# Autodesk Inventor assembly: TT_Tray
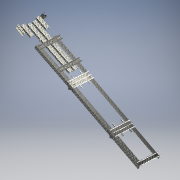
[picture p0: Inventor's stored thumbnail of the model, 180x180]
Saved by Autodesk Inventor 2019 (Build 230136000, 136)
## iProperties
Created: 2020-02-09
Part Number: TT_Tray
Document SubType Name: Assembly
Designer: samue
Author: samue
## Documents named in this file (25)
- C:\Users\samue\OneDrive\Desktop\CAD\TT_Tray.iam
- C:\Users\samue\OneDrive\Desktop\SID Library-20181221T043518Z-001\2018 BNS-VRC-SID Library\Structure\C-Channels\C-Channel 1x2x1\Aluminum C-Channel 1x2x1x30.ipt
- C:\Users\samue\OneDrive\Desktop\SID Library-20181221T043518Z-001\2018 BNS-VRC-SID Library\Structure\Standoffs _ Couplers\Standoff 0.50_.ipt
- C:\Users\samue\OneDrive\Desktop\SID Library-20181221T043518Z-001\2018 BNS-VRC-SID Library\Structure\C-Channels\C-Channel 1x2x1\Aluminum C-Channel 1x2x1x7.ipt
- C:\Users\samue\OneDrive\Desktop\SID Library-20181221T043518Z-001\2018 BNS-VRC-SID Library\Structure\C-Channels\C-Channel 1x2x1\Aluminum C-Channel 1x2x1x12.ipt
- C:\Users\samue\OneDrive\Desktop\SID Library-20181221T043518Z-001\2018 BNS-VRC-SID Library\Motion\Bearing Flat.ipt
- C:\Users\samue\OneDrive\Desktop\SID Library-20181221T043518Z-001\2018 BNS-VRC-SID Library\Structure\Screws _ Nuts\Screw 8-32 x 0.750_.ipt
- C:\Users\samue\OneDrive\Desktop\SID Library-20181221T043518Z-001\2018 BNS-VRC-SID Library\Structure\Screws _ Nuts\Screw 8-32 x 0.500_.ipt
- C:\Users\samue\OneDrive\Desktop\SID Library-20181221T043518Z-001\2018 BNS-VRC-SID Library\Structure\C-Channels\C-Channel 1x2x1\Aluminum C-Channel 1x2x1x5.ipt
- C:\Users\samue\OneDrive\Desktop\SID Library-20181221T043518Z-001\2018 BNS-VRC-SID Library\Structure\Screws _ Nuts\8-32 Nylon-Insert Thin Hex Locknut.iam
- C:\Users\samue\OneDrive\Desktop\SID Library-20181221T043518Z-001\2018 BNS-VRC-SID Library\Motion\Washers _ Spacers\Spacer (Nylon), 0.125_.ipt
- C:\Users\samue\OneDrive\Desktop\SID Library-20181221T043518Z-001\2018 BNS-VRC-SID Library\Motion\Washers _ Spacers\Washer, Steel, 0.032_.ipt
- C:\Users\samue\OneDrive\Desktop\SID Library-20181221T043518Z-001\2018 BNS-VRC-SID Library\Structure\Screws _ Nuts\Screw 8-32 x 1.250_.ipt
- C:\Users\samue\OneDrive\Desktop\SID Library-20181221T043518Z-001\2018 BNS-VRC-SID Library\Motion\Washers _ Spacers\Spacer (Nylon), 0.250_.ipt
- C:\Users\samue\OneDrive\Desktop\SID Library-20181221T043518Z-001\2018 BNS-VRC-SID Library\Structure\Screws _ Nuts\Screw 8-32 x 1.500_.ipt
- C:\Users\samue\OneDrive\Desktop\SID Library-20181221T043518Z-001\2018 BNS-VRC-SID Library\Structure\Screws _ Nuts\Nut 8-32 Keps.ipt
- C:\Users\samue\OneDrive\Desktop\SID Library-20181221T043518Z-001\2018 BNS-VRC-SID Library\Structure\Angles\Aluminum Angle\Aluminum Angle 2x2x25.ipt
- C:\Users\samue\OneDrive\Desktop\SID Library-20181221T043518Z-001\2018 BNS-VRC-SID Library\Motion\Washers _ Spacers\Spacer (Nylon), 0.500_.ipt
- C:\Users\samue\OneDrive\Desktop\SID Library-20181221T043518Z-001\2018 BNS-VRC-SID Library\Structure\Screws _ Nuts\8-32 Shoulder Screw.ipt
- C:\Users\samue\OneDrive\Desktop\SID Library-20181221T043518Z-001\2018 BNS-VRC-SID Library\Structure\Gussets\45 Degree Gusset.ipt
- C:\Users\samue\OneDrive\Desktop\SID Library-20181221T043518Z-001\2018 BNS-VRC-SID Library\Structure\Screws _ Nuts\Screw 8-32 x 0.375_.ipt
- C:\Users\samue\OneDrive\Desktop\SID Library-20181221T043518Z-001\2018 BNS-VRC-SID Library\Structure\C-Channels\C-Channel 1x2x1\Aluminum C-Channel 1x2x1x13.ipt
- C:\Users\samue\OneDrive\Desktop\SID Library-20181221T043518Z-001\2018 BNS-VRC-SID Library\Structure\Angles\Aluminum Angle\Aluminum Angle 2x2x20.ipt
- C:\Users\samue\OneDrive\Desktop\SID Library-20181221T043518Z-001\2018 BNS-VRC-SID Library\Structure\Standoffs _ Couplers\Standoff 1.00_.ipt
- C:\Users\samue\OneDrive\Desktop\SID Library-20181221T043518Z-001\2018 BNS-VRC-SID Library\Structure\Angles\Aluminum Angle\Aluminum Angle 2x2x30.ipt
## Components (213 placed, 24 different names)
1. Aluminum C-Channel 1x2x1x30:1 — Insert:1, Insert:16, Insert:76, Insert:78, Insert:81, Insert:85, Insert:87, Insert:89, Insert:99, Insert:104, Insert:106, Insert:108, Insert:109, Insert:112, Insert:116, Insert:118, Insert:119, Insert:132
2. Aluminum C-Channel 1x2x1x30:2 — Insert:2, Insert:14, Insert:79, Insert:80, Insert:83, Insert:86, Insert:88, Insert:90, Insert:98, Insert:105, Insert:107, Insert:110, Insert:111, Insert:113, Insert:117, Insert:120, Insert:121, Insert:133
3. Standoff 0.50_:1 — Insert:1, Insert:2
4. Aluminum C-Channel 1x2x1x7:1 — Insert:17, Insert:18, Insert:19, Insert:28, Insert:29, Insert:47, Insert:75
5. Aluminum C-Channel 1x2x1x7:2 — Insert:15, Insert:20, Insert:21, Insert:32, Insert:33, Insert:77
6. Standoff 0.50_:2 — Insert:14, Insert:15
7. Standoff 0.50_:3 — Insert:16, Insert:17
8. Bearing Flat:1 — Insert:18, Insert:19, Insert:49, Insert:71, Insert:72
9. Bearing Flat:2 — Insert:20, Insert:21, Insert:65, Insert:66, Insert:73, Insert:74
10. Screw 8-32 x 0.500_:5 — Insert:28
11. Screw 8-32 x 0.500_:6 — Insert:29
12. Screw 8-32 x 0.500_:7 — Insert:32
13. Screw 8-32 x 0.500_:8 — Insert:33
14. Aluminum C-Channel 1x2x1x5:1 — Insert:36, Insert:37, Insert:43, Insert:67, Insert:68
15. Bearing Flat:3 — Insert:36, Insert:37, Insert:48, Insert:69, Insert:70
16. 8-32 Nylon-Insert Thin Hex Locknut:1 [sub-assembly] — Insert:43, Insert:44
17. Spacer (Nylon), 0.125_:1 — Insert:44, Insert:45
18. Washer, Steel, 0.032_:1 — Insert:45, Insert:46
19. Washer, Steel, 0.032_:2 — Insert:46, Insert:47
20. Screw 8-32 x 1.250_:1 — Insert:48
21. 8-32 Nylon-Insert Thin Hex Locknut:2 [sub-assembly] — Insert:49
22. Aluminum C-Channel 1x2x1x5:2 — Insert:61, Insert:63
23. Bearing Flat:4 — Insert:60, Insert:62, Insert:64
24. 8-32 Nylon-Insert Thin Hex Locknut:3 [sub-assembly]
25. Spacer (Nylon), 0.125_:2
26. Washer, Steel, 0.032_:3
27. Washer, Steel, 0.032_:4 — Insert:65
28. Screw 8-32 x 1.250_:2 — Insert:60
29. Screw 8-32 x 0.500_:12 — Insert:61
30. 8-32 Nylon-Insert Thin Hex Locknut:4 [sub-assembly] — Insert:62
31. Screw 8-32 x 0.500_:13 — Insert:63
32. 8-32 Nylon-Insert Thin Hex Locknut:5 [sub-assembly] — Insert:64
33. 8-32 Nylon-Insert Thin Hex Locknut:6 [sub-assembly] — Insert:66
34. 8-32 Nylon-Insert Thin Hex Locknut:7 [sub-assembly] — Insert:70
35. 8-32 Nylon-Insert Thin Hex Locknut:8 [sub-assembly] — Insert:69
36. Screw 8-32 x 0.500_:14 — Insert:67
37. Screw 8-32 x 0.500_:15 — Insert:68
38. 8-32 Nylon-Insert Thin Hex Locknut:9 [sub-assembly] — Insert:71
39. 8-32 Nylon-Insert Thin Hex Locknut:10 [sub-assembly] — Insert:72
40. 8-32 Nylon-Insert Thin Hex Locknut:11 [sub-assembly] — Insert:73
41. 8-32 Nylon-Insert Thin Hex Locknut:12 [sub-assembly] — Insert:74
42. Screw 8-32 x 0.750_:1 — Insert:75
43. Screw 8-32 x 0.750_:2 — Insert:76
44. Screw 8-32 x 0.750_:3 — Insert:77
45. 8-32 Nylon-Insert Thin Hex Locknut:13 [sub-assembly] — Insert:78
46. 8-32 Nylon-Insert Thin Hex Locknut:14 [sub-assembly] — Insert:79
47. 8-32 Nylon-Insert Thin Hex Locknut:15 [sub-assembly] — Insert:80
48. Spacer (Nylon), 0.250_:1 — Insert:81, Insert:82
49. Screw 8-32 x 1.500_:1 — Insert:82
50. Spacer (Nylon), 0.250_:2 — Insert:83, Insert:84
51. Screw 8-32 x 1.500_:2 — Insert:84
52. Standoff 0.50_:4 — Insert:85, Insert:86
53. Nut 8-32 Keps:1 — Insert:87
54. Nut 8-32 Keps:2 — Insert:88
55. Nut 8-32 Keps:3 — Insert:90
56. Nut 8-32 Keps:4 — Insert:89
57. Aluminum Angle 2x2x25:1 — Insert:122, Insert:123, Insert:135, Insert:136, Insert:143, Insert:144, Insert:147, Insert:168, Insert:169, Insert:176, Insert:177, Insert:184, Insert:185, Insert:190, Insert:191
58. 8-32 Shoulder Screw:1 — Insert:98
59. 8-32 Shoulder Screw:2 — Insert:99
60. 8-32 Nylon-Insert Thin Hex Locknut:17 [sub-assembly]
61. 8-32 Nylon-Insert Thin Hex Locknut:18 [sub-assembly]
62. Standoff 0.50_:5 — Insert:104, Insert:105
63. Screw 8-32 x 0.750_:6 — Insert:106
64. 8-32 Nylon-Insert Thin Hex Locknut:20 [sub-assembly] — Insert:107
65. Screw 8-32 x 0.500_:16 — Insert:108
66. Screw 8-32 x 0.500_:17 — Insert:109
67. Screw 8-32 x 0.500_:18 — Insert:110
68. Screw 8-32 x 0.500_:19 — Insert:111
69. Screw 8-32 x 1.500_:3 — Insert:114
70. Spacer (Nylon), 0.250_:3 — Insert:112, Insert:114
71. Spacer (Nylon), 0.250_:4 — Insert:113, Insert:115
72. Screw 8-32 x 1.500_:4 — Insert:115
73. Standoff 0.50_:6 — Insert:116, Insert:117
74. Nut 8-32 Keps:5 — Insert:118
75. Nut 8-32 Keps:6 — Insert:119
76. Nut 8-32 Keps:7 — Insert:120
77. Nut 8-32 Keps:8 — Insert:121
78. Spacer (Nylon), 0.500_:3 — Insert:123, Insert:158
79. Spacer (Nylon), 0.500_:4 — Insert:122, Insert:159
80. 8-32 Nylon-Insert Thin Hex Locknut:21 [sub-assembly] — Insert:164
81. 8-32 Shoulder Screw:3 — Insert:132
82. 8-32 Shoulder Screw:4 — Insert:133
83. Screw 8-32 x 0.750_:7 — Insert:135
84. Screw 8-32 x 0.750_:8 — Insert:136
85. 45 Degree Gusset:1 — Insert:143, Insert:144, Insert:145, Insert:146, Insert:239, Insert:257
86. Screw 8-32 x 0.375_:1 — Insert:146
87. Screw 8-32 x 0.375_:2 — Insert:145
88. Aluminum C-Channel 1x2x1x12:2 — Insert:147, Insert:148, Insert:149, Insert:186, Insert:187, Insert:188, Insert:189, Insert:235, Insert:236
89. Aluminum Angle 2x2x25:2 — Insert:148, Insert:149, Insert:152, Insert:153, Insert:154, Insert:155, Insert:166, Insert:167, Insert:174, Insert:175, Insert:182, Insert:183, Insert:192, Insert:193, Insert:196, Insert:197
90. Screw 8-32 x 0.750_:11 — Insert:174
91. Spacer (Nylon), 0.500_:7 — Insert:166, Insert:170
92. Screw 8-32 x 0.750_:12 — Insert:152
93. Screw 8-32 x 0.750_:13 — Insert:153
94. Spacer (Nylon), 0.500_:8 — Insert:155, Insert:156
95. Spacer (Nylon), 0.500_:9 — Insert:154, Insert:157
96. Aluminum C-Channel 1x2x1x13:1 — Insert:156, Insert:157, Insert:158, Insert:159, Insert:160, Insert:161, Insert:162, Insert:163, Insert:164, Insert:165
97. 8-32 Nylon-Insert Thin Hex Locknut:28 [sub-assembly] — Insert:160
98. 8-32 Nylon-Insert Thin Hex Locknut:29 [sub-assembly] — Insert:161
99. 8-32 Nylon-Insert Thin Hex Locknut:30 [sub-assembly] — Insert:163
100. 8-32 Nylon-Insert Thin Hex Locknut:31 [sub-assembly] — Insert:162
101. 8-32 Nylon-Insert Thin Hex Locknut:32 [sub-assembly] — Insert:165
102. Aluminum C-Channel 1x2x1x13:2 — Insert:170, Insert:171, Insert:172, Insert:173, Insert:178, Insert:179, Insert:180, Insert:181
103. Spacer (Nylon), 0.500_:10 — Insert:167, Insert:171
104. Spacer (Nylon), 0.500_:11 — Insert:169, Insert:173
105. Spacer (Nylon), 0.500_:12 — Insert:168, Insert:172
106. Screw 8-32 x 0.750_:14 — Insert:175
107. Screw 8-32 x 0.750_:15 — Insert:176
108. Screw 8-32 x 0.750_:16 — Insert:177
109. 8-32 Nylon-Insert Thin Hex Locknut:33 [sub-assembly] — Insert:178
110. 8-32 Nylon-Insert Thin Hex Locknut:34 [sub-assembly] — Insert:179
111. 8-32 Nylon-Insert Thin Hex Locknut:35 [sub-assembly] — Insert:180
112. 8-32 Nylon-Insert Thin Hex Locknut:36 [sub-assembly] — Insert:181
113. Screw 8-32 x 0.375_:3 — Insert:182
114. Screw 8-32 x 0.375_:4 — Insert:183
115. Screw 8-32 x 0.375_:5 — Insert:184
116. Screw 8-32 x 0.375_:6 — Insert:185
117. 8-32 Nylon-Insert Thin Hex Locknut:37 [sub-assembly] — Insert:186
118. 8-32 Nylon-Insert Thin Hex Locknut:38 [sub-assembly] — Insert:187
119. 8-32 Nylon-Insert Thin Hex Locknut:39 [sub-assembly] — Insert:188
120. 8-32 Nylon-Insert Thin Hex Locknut:40 [sub-assembly] — Insert:189
121. 8-32 Nylon-Insert Thin Hex Locknut:41 [sub-assembly] — Insert:190
122. 8-32 Nylon-Insert Thin Hex Locknut:42 [sub-assembly] — Insert:191
123. 45 Degree Gusset:2 — Insert:192, Insert:193, Insert:194, Insert:195, Insert:246, Insert:259
124. Screw 8-32 x 0.375_:7 — Insert:195
125. Screw 8-32 x 0.375_:8 — Insert:194
126. 8-32 Nylon-Insert Thin Hex Locknut:43 [sub-assembly] — Insert:196
127. 8-32 Nylon-Insert Thin Hex Locknut:44 [sub-assembly] — Insert:197
128. 45 Degree Gusset:3 — Insert:206, Insert:207, Insert:216, Insert:217, Insert:285, Insert:295
129. 45 Degree Gusset:4 — Insert:208, Insert:209, Insert:218, Insert:219, Insert:288, Insert:298
130. Aluminum Angle 2x2x20:1 — Insert:206, Insert:207, Insert:212, Insert:213, Insert:220, Insert:221, Insert:225, Insert:231, Insert:317, Insert:318
131. Aluminum Angle 2x2x20:2 — Insert:208, Insert:209, Insert:214, Insert:215, Insert:222, Insert:226, Insert:232, Insert:319, Insert:320
132. Screw 8-32 x 0.375_:11 — Insert:212
133. Screw 8-32 x 0.375_:12 — Insert:213
134. Screw 8-32 x 0.375_:13 — Insert:214
135. Screw 8-32 x 0.375_:14 — Insert:215
136. 8-32 Nylon-Insert Thin Hex Locknut:47 [sub-assembly] — Insert:216
137. 8-32 Nylon-Insert Thin Hex Locknut:48 [sub-assembly] — Insert:217
138. 8-32 Nylon-Insert Thin Hex Locknut:49 [sub-assembly] — Insert:218
139. 8-32 Nylon-Insert Thin Hex Locknut:50 [sub-assembly] — Insert:219
140. Aluminum C-Channel 1x2x1x12:3 — Insert:220, Insert:221, Insert:222, Insert:227, Insert:228, Insert:229, Insert:230, Insert:233, Insert:234
141. Screw 8-32 x 0.375_:15 — Insert:226
142. Screw 8-32 x 0.375_:16 — Insert:225
143. 8-32 Nylon-Insert Thin Hex Locknut:51 [sub-assembly] — Insert:227
144. 8-32 Nylon-Insert Thin Hex Locknut:52 [sub-assembly] — Insert:228
145. 8-32 Nylon-Insert Thin Hex Locknut:53 [sub-assembly] — Insert:229
146. 8-32 Nylon-Insert Thin Hex Locknut:54 [sub-assembly] — Insert:230
147. 8-32 Shoulder Screw:6 — Insert:231
148. 8-32 Shoulder Screw:7 — Insert:232
149. Standoff 1.00_:1 — Insert:233
150. Standoff 1.00_:2 — Insert:234
151. Standoff 1.00_:3 — Insert:236
152. Standoff 1.00_:4 — Insert:235
153. Aluminum Angle 2x2x30:1 — Insert:237, Insert:238, Insert:249, Insert:250, Insert:265, Insert:266, Insert:269, Insert:270, Insert:279, Insert:280, Insert:296, Insert:297, Insert:301, Insert:302, Insert:305, Insert:308
154. Aluminum Angle 2x2x30:2 — Insert:244, Insert:245, Insert:251, Insert:252, Insert:263, Insert:264, Insert:267, Insert:268, Insert:283, Insert:284, Insert:299, Insert:300, Insert:303, Insert:304, Insert:306, Insert:307
155. 45 Degree Gusset:5 — Insert:237, Insert:238, Insert:241, Insert:253, Insert:254, Insert:258
156. Washer, Steel, 0.032_:5 — Insert:240, Insert:241
157. Washer, Steel, 0.032_:6 — Insert:239, Insert:240
158. 45 Degree Gusset:6 — Insert:244, Insert:245, Insert:248, Insert:255, Insert:256, Insert:260
159. Washer, Steel, 0.032_:7 — Insert:246, Insert:247
160. Washer, Steel, 0.032_:8 — Insert:247, Insert:248
161. Screw 8-32 x 0.375_:17 — Insert:249
162. Screw 8-32 x 0.375_:18 — Insert:250
163. Screw 8-32 x 0.375_:19 — Insert:251
164. Screw 8-32 x 0.375_:20 — Insert:252
165. 8-32 Nylon-Insert Thin Hex Locknut:55 [sub-assembly] — Insert:253
166. 8-32 Nylon-Insert Thin Hex Locknut:56 [sub-assembly] — Insert:254
167. 8-32 Nylon-Insert Thin Hex Locknut:57 [sub-assembly] — Insert:255
168. 8-32 Nylon-Insert Thin Hex Locknut:58 [sub-assembly] — Insert:256
169. Screw 8-32 x 0.375_:21 — Insert:257
170. 8-32 Nylon-Insert Thin Hex Locknut:59 [sub-assembly] — Insert:258
171. Screw 8-32 x 0.375_:22 — Insert:259
172. 8-32 Nylon-Insert Thin Hex Locknut:60 [sub-assembly] — Insert:260
173. Aluminum C-Channel 1x2x1x12:4 — Insert:263, Insert:264, Insert:265, Insert:266, Insert:273, Insert:274, Insert:313, Insert:314, Insert:315, Insert:316
174. Standoff 1.00_:5 — Insert:271
175. Standoff 1.00_:6 — Insert:272
176. Aluminum C-Channel 1x2x1x12:5 — Insert:267, Insert:268, Insert:269, Insert:270, Insert:271, Insert:272, Insert:309, Insert:310, Insert:311, Insert:312
177. Standoff 1.00_:7 — Insert:274
178. Standoff 1.00_:8 — Insert:273
179. Washer, Steel, 0.032_:9 — Insert:281, Insert:282
180. Washer, Steel, 0.032_:10 — Insert:282, Insert:285
181. 45 Degree Gusset:9 — Insert:279, Insert:280, Insert:281, Insert:289, Insert:290, Insert:294
182. 45 Degree Gusset:10 — Insert:283, Insert:284, Insert:286, Insert:291, Insert:292, Insert:293
183. Washer, Steel, 0.032_:11 — Insert:286, Insert:287
184. Washer, Steel, 0.032_:12 — Insert:287, Insert:288
185. Screw 8-32 x 0.375_:23 — Insert:289
186. Screw 8-32 x 0.375_:24 — Insert:290
187. Screw 8-32 x 0.375_:25 — Insert:291
188. Screw 8-32 x 0.375_:26 — Insert:292
189. Screw 8-32 x 0.375_:27 — Insert:293
190. Screw 8-32 x 0.375_:28 — Insert:294
191. 8-32 Nylon-Insert Thin Hex Locknut:61 [sub-assembly] — Insert:295
192. 8-32 Nylon-Insert Thin Hex Locknut:62 [sub-assembly] — Insert:296
193. 8-32 Nylon-Insert Thin Hex Locknut:63 [sub-assembly] — Insert:297
194. 8-32 Nylon-Insert Thin Hex Locknut:64 [sub-assembly] — Insert:298
195. 8-32 Nylon-Insert Thin Hex Locknut:65 [sub-assembly] — Insert:299
196. 8-32 Nylon-Insert Thin Hex Locknut:66 [sub-assembly] — Insert:300
197. Screw 8-32 x 0.375_:29 — Insert:301
198. Screw 8-32 x 0.375_:30 — Insert:302
199. Screw 8-32 x 0.375_:31 — Insert:303
200. Screw 8-32 x 0.375_:32 — Insert:304
201. 8-32 Shoulder Screw:8 — Insert:305
202. 8-32 Shoulder Screw:9 — Insert:306
203. Screw 8-32 x 0.375_:33 — Insert:307
204. Screw 8-32 x 0.375_:34 — Insert:308
205. 8-32 Nylon-Insert Thin Hex Locknut:67 [sub-assembly] — Insert:309
206. 8-32 Nylon-Insert Thin Hex Locknut:68 [sub-assembly] — Insert:310
207. 8-32 Nylon-Insert Thin Hex Locknut:69 [sub-assembly] — Insert:311
208. 8-32 Nylon-Insert Thin Hex Locknut:70 [sub-assembly] — Insert:312
209. 8-32 Nylon-Insert Thin Hex Locknut:71 [sub-assembly] — Insert:313
210. 8-32 Nylon-Insert Thin Hex Locknut:72 [sub-assembly] — Insert:314
211. 8-32 Nylon-Insert Thin Hex Locknut:73 [sub-assembly] — Insert:315
212. 8-32 Nylon-Insert Thin Hex Locknut:74 [sub-assembly] — Insert:316
213. Aluminum C-Channel 1x2x1x12:6 — Insert:317, Insert:318, Insert:319, Insert:320
## Relationships (242: Insert 242)
- Insert:1: Aluminum C-Channel 1x2x1x30:1 ↔ Standoff 0.50_:1
- Insert:2: Aluminum C-Channel 1x2x1x30:2 ↔ Standoff 0.50_:1
- Insert:14: Aluminum C-Channel 1x2x1x30:2 ↔ Standoff 0.50_:2
- Insert:15: Aluminum C-Channel 1x2x1x7:2 ↔ Standoff 0.50_:2
- Insert:16: Aluminum C-Channel 1x2x1x30:1 ↔ Standoff 0.50_:3
- Insert:17: Aluminum C-Channel 1x2x1x7:1 ↔ Standoff 0.50_:3
- Insert:18: Aluminum C-Channel 1x2x1x7:1 ↔ Bearing Flat:1
- Insert:19: Aluminum C-Channel 1x2x1x7:1 ↔ Bearing Flat:1
- Insert:20: Aluminum C-Channel 1x2x1x7:2 ↔ Bearing Flat:2
- Insert:21: Aluminum C-Channel 1x2x1x7:2 ↔ Bearing Flat:2
- Insert:28: Aluminum C-Channel 1x2x1x7:1 ↔ Screw 8-32 x 0.500_:5
- Insert:29: Aluminum C-Channel 1x2x1x7:1 ↔ Screw 8-32 x 0.500_:6
- Insert:32: Aluminum C-Channel 1x2x1x7:2 ↔ Screw 8-32 x 0.500_:7
- Insert:33: Aluminum C-Channel 1x2x1x7:2 ↔ Screw 8-32 x 0.500_:8
- Insert:36: Aluminum C-Channel 1x2x1x5:1 ↔ Bearing Flat:3
- Insert:37: Aluminum C-Channel 1x2x1x5:1 ↔ Bearing Flat:3
- Insert:43: Aluminum C-Channel 1x2x1x5:1 ↔ 8-32 Nylon-Insert Thin Hex Locknut:1
- Insert:44: 8-32 Nylon-Insert Thin Hex Locknut:1 ↔ Spacer (Nylon), 0.125_:1
- Insert:45: Spacer (Nylon), 0.125_:1 ↔ Washer, Steel, 0.032_:1
- Insert:46: Washer, Steel, 0.032_:1 ↔ Washer, Steel, 0.032_:2
- Insert:47: Aluminum C-Channel 1x2x1x7:1 ↔ Washer, Steel, 0.032_:2
- Insert:48: Bearing Flat:3 ↔ Screw 8-32 x 1.250_:1
- Insert:49: Bearing Flat:1 ↔ 8-32 Nylon-Insert Thin Hex Locknut:2
- [Insert]: Aluminum C-Channel 1x2x1x5:2 ↔ Bearing Flat:4
- [Insert]: Aluminum C-Channel 1x2x1x5:2 ↔ Bearing Flat:4
- [Insert]: Aluminum C-Channel 1x2x1x5:2 ↔ 8-32 Nylon-Insert Thin Hex Locknut:3
- [Insert]: 8-32 Nylon-Insert Thin Hex Locknut:3 ↔ Spacer (Nylon), 0.125_:2
- [Insert]: Spacer (Nylon), 0.125_:2 ↔ Washer, Steel, 0.032_:3
- [Insert]: Washer, Steel, 0.032_:3 ↔ Washer, Steel, 0.032_:4
- Insert:60: Bearing Flat:4 ↔ Screw 8-32 x 1.250_:2
- Insert:61: Aluminum C-Channel 1x2x1x5:2 ↔ Screw 8-32 x 0.500_:12
- Insert:62: Bearing Flat:4 ↔ 8-32 Nylon-Insert Thin Hex Locknut:4
- Insert:63: Aluminum C-Channel 1x2x1x5:2 ↔ Screw 8-32 x 0.500_:13
- Insert:64: Bearing Flat:4 ↔ 8-32 Nylon-Insert Thin Hex Locknut:5
- Insert:65: Bearing Flat:2 ↔ Washer, Steel, 0.032_:4
- Insert:66: Bearing Flat:2 ↔ 8-32 Nylon-Insert Thin Hex Locknut:6
- Insert:67: Aluminum C-Channel 1x2x1x5:1 ↔ Screw 8-32 x 0.500_:14
- Insert:68: Aluminum C-Channel 1x2x1x5:1 ↔ Screw 8-32 x 0.500_:15
- Insert:69: Bearing Flat:3 ↔ 8-32 Nylon-Insert Thin Hex Locknut:8
- Insert:70: Bearing Flat:3 ↔ 8-32 Nylon-Insert Thin Hex Locknut:7
- Insert:71: Bearing Flat:1 ↔ 8-32 Nylon-Insert Thin Hex Locknut:9
- Insert:72: Bearing Flat:1 ↔ 8-32 Nylon-Insert Thin Hex Locknut:10
- Insert:73: Bearing Flat:2 ↔ 8-32 Nylon-Insert Thin Hex Locknut:11
- Insert:74: Bearing Flat:2 ↔ 8-32 Nylon-Insert Thin Hex Locknut:12
- Insert:75: Aluminum C-Channel 1x2x1x7:1 ↔ Screw 8-32 x 0.750_:1
- Insert:76: Aluminum C-Channel 1x2x1x30:1 ↔ Screw 8-32 x 0.750_:2
- Insert:77: Aluminum C-Channel 1x2x1x7:2 ↔ Screw 8-32 x 0.750_:3
- Insert:78: Aluminum C-Channel 1x2x1x30:1 ↔ 8-32 Nylon-Insert Thin Hex Locknut:13
- Insert:79: Aluminum C-Channel 1x2x1x30:2 ↔ 8-32 Nylon-Insert Thin Hex Locknut:14
- Insert:80: Aluminum C-Channel 1x2x1x30:2 ↔ 8-32 Nylon-Insert Thin Hex Locknut:15
- Insert:81: Aluminum C-Channel 1x2x1x30:1 ↔ Spacer (Nylon), 0.250_:1
- Insert:82: Spacer (Nylon), 0.250_:1 ↔ Screw 8-32 x 1.500_:1
- Insert:83: Aluminum C-Channel 1x2x1x30:2 ↔ Spacer (Nylon), 0.250_:2
- Insert:84: Spacer (Nylon), 0.250_:2 ↔ Screw 8-32 x 1.500_:2
- Insert:85: Aluminum C-Channel 1x2x1x30:1 ↔ Standoff 0.50_:4
- Insert:86: Aluminum C-Channel 1x2x1x30:2 ↔ Standoff 0.50_:4
- Insert:87: Aluminum C-Channel 1x2x1x30:1 ↔ Nut 8-32 Keps:1
- Insert:88: Aluminum C-Channel 1x2x1x30:2 ↔ Nut 8-32 Keps:2
- Insert:89: Aluminum C-Channel 1x2x1x30:1 ↔ Nut 8-32 Keps:4
- Insert:90: Aluminum C-Channel 1x2x1x30:2 ↔ Nut 8-32 Keps:3
- Insert:98: Aluminum C-Channel 1x2x1x30:2 ↔ 8-32 Shoulder Screw:1
- Insert:99: Aluminum C-Channel 1x2x1x30:1 ↔ 8-32 Shoulder Screw:2
- Insert:104: Aluminum C-Channel 1x2x1x30:1 ↔ Standoff 0.50_:5
- Insert:105: Aluminum C-Channel 1x2x1x30:2 ↔ Standoff 0.50_:5
- Insert:106: Aluminum C-Channel 1x2x1x30:1 ↔ Screw 8-32 x 0.750_:6
- Insert:107: Aluminum C-Channel 1x2x1x30:2 ↔ 8-32 Nylon-Insert Thin Hex Locknut:20
- Insert:108: Aluminum C-Channel 1x2x1x30:1 ↔ Screw 8-32 x 0.500_:16
- Insert:109: Aluminum C-Channel 1x2x1x30:1 ↔ Screw 8-32 x 0.500_:17
- Insert:110: Aluminum C-Channel 1x2x1x30:2 ↔ Screw 8-32 x 0.500_:18
- Insert:111: Aluminum C-Channel 1x2x1x30:2 ↔ Screw 8-32 x 0.500_:19
- Insert:112: Aluminum C-Channel 1x2x1x30:1 ↔ Spacer (Nylon), 0.250_:3
- Insert:113: Aluminum C-Channel 1x2x1x30:2 ↔ Spacer (Nylon), 0.250_:4
- Insert:114: Screw 8-32 x 1.500_:3 ↔ Spacer (Nylon), 0.250_:3
- Insert:115: Spacer (Nylon), 0.250_:4 ↔ Screw 8-32 x 1.500_:4
- Insert:116: Aluminum C-Channel 1x2x1x30:1 ↔ Standoff 0.50_:6
- Insert:117: Aluminum C-Channel 1x2x1x30:2 ↔ Standoff 0.50_:6
- Insert:118: Aluminum C-Channel 1x2x1x30:1 ↔ Nut 8-32 Keps:5
- Insert:119: Aluminum C-Channel 1x2x1x30:1 ↔ Nut 8-32 Keps:6
- Insert:120: Aluminum C-Channel 1x2x1x30:2 ↔ Nut 8-32 Keps:7
- Insert:121: Aluminum C-Channel 1x2x1x30:2 ↔ Nut 8-32 Keps:8
- Insert:122: Aluminum Angle 2x2x25:1 ↔ Spacer (Nylon), 0.500_:4
- Insert:123: Aluminum Angle 2x2x25:1 ↔ Spacer (Nylon), 0.500_:3
- Insert:132: Aluminum C-Channel 1x2x1x30:1 ↔ 8-32 Shoulder Screw:3
- Insert:133: Aluminum C-Channel 1x2x1x30:2 ↔ 8-32 Shoulder Screw:4
- Insert:135: Aluminum Angle 2x2x25:1 ↔ Screw 8-32 x 0.750_:7
- Insert:136: Aluminum Angle 2x2x25:1 ↔ Screw 8-32 x 0.750_:8
- Insert:143: Aluminum Angle 2x2x25:1 ↔ 45 Degree Gusset:1
- Insert:144: Aluminum Angle 2x2x25:1 ↔ 45 Degree Gusset:1
- Insert:145: 45 Degree Gusset:1 ↔ Screw 8-32 x 0.375_:2
- Insert:146: 45 Degree Gusset:1 ↔ Screw 8-32 x 0.375_:1
- Insert:147: Aluminum Angle 2x2x25:1 ↔ Aluminum C-Channel 1x2x1x12:2
- Insert:148: Aluminum C-Channel 1x2x1x12:2 ↔ Aluminum Angle 2x2x25:2
- Insert:149: Aluminum C-Channel 1x2x1x12:2 ↔ Aluminum Angle 2x2x25:2
- Insert:152: Aluminum Angle 2x2x25:2 ↔ Screw 8-32 x 0.750_:12
- Insert:153: Aluminum Angle 2x2x25:2 ↔ Screw 8-32 x 0.750_:13
- Insert:154: Aluminum Angle 2x2x25:2 ↔ Spacer (Nylon), 0.500_:9
- Insert:155: Aluminum Angle 2x2x25:2 ↔ Spacer (Nylon), 0.500_:8
- Insert:156: Spacer (Nylon), 0.500_:8 ↔ Aluminum C-Channel 1x2x1x13:1
- Insert:157: Spacer (Nylon), 0.500_:9 ↔ Aluminum C-Channel 1x2x1x13:1
- Insert:158: Spacer (Nylon), 0.500_:3 ↔ Aluminum C-Channel 1x2x1x13:1
- Insert:159: Spacer (Nylon), 0.500_:4 ↔ Aluminum C-Channel 1x2x1x13:1
- Insert:160: Aluminum C-Channel 1x2x1x13:1 ↔ 8-32 Nylon-Insert Thin Hex Locknut:28
- Insert:161: Aluminum C-Channel 1x2x1x13:1 ↔ 8-32 Nylon-Insert Thin Hex Locknut:29
- Insert:162: Aluminum C-Channel 1x2x1x13:1 ↔ 8-32 Nylon-Insert Thin Hex Locknut:31
- Insert:163: Aluminum C-Channel 1x2x1x13:1 ↔ 8-32 Nylon-Insert Thin Hex Locknut:30
- Insert:164: 8-32 Nylon-Insert Thin Hex Locknut:21 ↔ Aluminum C-Channel 1x2x1x13:1
- Insert:165: Aluminum C-Channel 1x2x1x13:1 ↔ 8-32 Nylon-Insert Thin Hex Locknut:32
- Insert:166: Aluminum Angle 2x2x25:2 ↔ Spacer (Nylon), 0.500_:7
- Insert:167: Aluminum Angle 2x2x25:2 ↔ Spacer (Nylon), 0.500_:10
- Insert:168: Aluminum Angle 2x2x25:1 ↔ Spacer (Nylon), 0.500_:12
- Insert:169: Aluminum Angle 2x2x25:1 ↔ Spacer (Nylon), 0.500_:11
- Insert:170: Spacer (Nylon), 0.500_:7 ↔ Aluminum C-Channel 1x2x1x13:2
- Insert:171: Aluminum C-Channel 1x2x1x13:2 ↔ Spacer (Nylon), 0.500_:10
- Insert:172: Aluminum C-Channel 1x2x1x13:2 ↔ Spacer (Nylon), 0.500_:12
- Insert:173: Aluminum C-Channel 1x2x1x13:2 ↔ Spacer (Nylon), 0.500_:11
- Insert:174: Aluminum Angle 2x2x25:2 ↔ Screw 8-32 x 0.750_:11
- Insert:175: Aluminum Angle 2x2x25:2 ↔ Screw 8-32 x 0.750_:14
- Insert:176: Aluminum Angle 2x2x25:1 ↔ Screw 8-32 x 0.750_:15
- Insert:177: Aluminum Angle 2x2x25:1 ↔ Screw 8-32 x 0.750_:16
- Insert:178: Aluminum C-Channel 1x2x1x13:2 ↔ 8-32 Nylon-Insert Thin Hex Locknut:33
- Insert:179: Aluminum C-Channel 1x2x1x13:2 ↔ 8-32 Nylon-Insert Thin Hex Locknut:34
- Insert:180: Aluminum C-Channel 1x2x1x13:2 ↔ 8-32 Nylon-Insert Thin Hex Locknut:35
- Insert:181: Aluminum C-Channel 1x2x1x13:2 ↔ 8-32 Nylon-Insert Thin Hex Locknut:36
- Insert:182: Aluminum Angle 2x2x25:2 ↔ Screw 8-32 x 0.375_:3
- Insert:183: Aluminum Angle 2x2x25:2 ↔ Screw 8-32 x 0.375_:4
- Insert:184: Aluminum Angle 2x2x25:1 ↔ Screw 8-32 x 0.375_:5
- Insert:185: Aluminum Angle 2x2x25:1 ↔ Screw 8-32 x 0.375_:6
- Insert:186: Aluminum C-Channel 1x2x1x12:2 ↔ 8-32 Nylon-Insert Thin Hex Locknut:37
- Insert:187: Aluminum C-Channel 1x2x1x12:2 ↔ 8-32 Nylon-Insert Thin Hex Locknut:38
- Insert:188: Aluminum C-Channel 1x2x1x12:2 ↔ 8-32 Nylon-Insert Thin Hex Locknut:39
- Insert:189: Aluminum C-Channel 1x2x1x12:2 ↔ 8-32 Nylon-Insert Thin Hex Locknut:40
- Insert:190: Aluminum Angle 2x2x25:1 ↔ 8-32 Nylon-Insert Thin Hex Locknut:41
- Insert:191: Aluminum Angle 2x2x25:1 ↔ 8-32 Nylon-Insert Thin Hex Locknut:42
- Insert:192: Aluminum Angle 2x2x25:2 ↔ 45 Degree Gusset:2
- Insert:193: Aluminum Angle 2x2x25:2 ↔ 45 Degree Gusset:2
- Insert:194: 45 Degree Gusset:2 ↔ Screw 8-32 x 0.375_:8
- Insert:195: 45 Degree Gusset:2 ↔ Screw 8-32 x 0.375_:7
- Insert:196: Aluminum Angle 2x2x25:2 ↔ 8-32 Nylon-Insert Thin Hex Locknut:43
- Insert:197: Aluminum Angle 2x2x25:2 ↔ 8-32 Nylon-Insert Thin Hex Locknut:44
- Insert:206: 45 Degree Gusset:3 ↔ Aluminum Angle 2x2x20:1
- Insert:207: 45 Degree Gusset:3 ↔ Aluminum Angle 2x2x20:1
- Insert:208: 45 Degree Gusset:4 ↔ Aluminum Angle 2x2x20:2
- Insert:209: 45 Degree Gusset:4 ↔ Aluminum Angle 2x2x20:2
- Insert:212: Aluminum Angle 2x2x20:1 ↔ Screw 8-32 x 0.375_:11
- Insert:213: Aluminum Angle 2x2x20:1 ↔ Screw 8-32 x 0.375_:12
- Insert:214: Aluminum Angle 2x2x20:2 ↔ Screw 8-32 x 0.375_:13
- Insert:215: Aluminum Angle 2x2x20:2 ↔ Screw 8-32 x 0.375_:14
- Insert:216: 45 Degree Gusset:3 ↔ 8-32 Nylon-Insert Thin Hex Locknut:47
- Insert:217: 45 Degree Gusset:3 ↔ 8-32 Nylon-Insert Thin Hex Locknut:48
- Insert:218: 45 Degree Gusset:4 ↔ 8-32 Nylon-Insert Thin Hex Locknut:49
- Insert:219: 45 Degree Gusset:4 ↔ 8-32 Nylon-Insert Thin Hex Locknut:50
- Insert:220: Aluminum Angle 2x2x20:1 ↔ Aluminum C-Channel 1x2x1x12:3
- Insert:221: Aluminum Angle 2x2x20:1 ↔ Aluminum C-Channel 1x2x1x12:3
- Insert:222: Aluminum Angle 2x2x20:2 ↔ Aluminum C-Channel 1x2x1x12:3
- Insert:225: Aluminum Angle 2x2x20:1 ↔ Screw 8-32 x 0.375_:16
- Insert:226: Aluminum Angle 2x2x20:2 ↔ Screw 8-32 x 0.375_:15
- Insert:227: Aluminum C-Channel 1x2x1x12:3 ↔ 8-32 Nylon-Insert Thin Hex Locknut:51
- Insert:228: Aluminum C-Channel 1x2x1x12:3 ↔ 8-32 Nylon-Insert Thin Hex Locknut:52
- Insert:229: Aluminum C-Channel 1x2x1x12:3 ↔ 8-32 Nylon-Insert Thin Hex Locknut:53
- Insert:230: Aluminum C-Channel 1x2x1x12:3 ↔ 8-32 Nylon-Insert Thin Hex Locknut:54
- Insert:231: Aluminum Angle 2x2x20:1 ↔ 8-32 Shoulder Screw:6
- Insert:232: Aluminum Angle 2x2x20:2 ↔ 8-32 Shoulder Screw:7
- Insert:233: Aluminum C-Channel 1x2x1x12:3 ↔ Standoff 1.00_:1
- Insert:234: Aluminum C-Channel 1x2x1x12:3 ↔ Standoff 1.00_:2
- Insert:235: Aluminum C-Channel 1x2x1x12:2 ↔ Standoff 1.00_:4
- Insert:236: Aluminum C-Channel 1x2x1x12:2 ↔ Standoff 1.00_:3
- Insert:237: Aluminum Angle 2x2x30:1 ↔ 45 Degree Gusset:5
- Insert:238: Aluminum Angle 2x2x30:1 ↔ 45 Degree Gusset:5
- Insert:239: 45 Degree Gusset:1 ↔ Washer, Steel, 0.032_:6
- Insert:240: Washer, Steel, 0.032_:5 ↔ Washer, Steel, 0.032_:6
- Insert:241: 45 Degree Gusset:5 ↔ Washer, Steel, 0.032_:5
- Insert:244: Aluminum Angle 2x2x30:2 ↔ 45 Degree Gusset:6
- Insert:245: Aluminum Angle 2x2x30:2 ↔ 45 Degree Gusset:6
- Insert:246: 45 Degree Gusset:2 ↔ Washer, Steel, 0.032_:7
- Insert:247: Washer, Steel, 0.032_:7 ↔ Washer, Steel, 0.032_:8
- Insert:248: 45 Degree Gusset:6 ↔ Washer, Steel, 0.032_:8
- Insert:249: Aluminum Angle 2x2x30:1 ↔ Screw 8-32 x 0.375_:17
- Insert:250: Aluminum Angle 2x2x30:1 ↔ Screw 8-32 x 0.375_:18
- Insert:251: Aluminum Angle 2x2x30:2 ↔ Screw 8-32 x 0.375_:19
- Insert:252: Aluminum Angle 2x2x30:2 ↔ Screw 8-32 x 0.375_:20
- Insert:253: 45 Degree Gusset:5 ↔ 8-32 Nylon-Insert Thin Hex Locknut:55
- Insert:254: 45 Degree Gusset:5 ↔ 8-32 Nylon-Insert Thin Hex Locknut:56
- Insert:255: 45 Degree Gusset:6 ↔ 8-32 Nylon-Insert Thin Hex Locknut:57
- Insert:256: 45 Degree Gusset:6 ↔ 8-32 Nylon-Insert Thin Hex Locknut:58
- Insert:257: 45 Degree Gusset:1 ↔ Screw 8-32 x 0.375_:21
- Insert:258: 45 Degree Gusset:5 ↔ 8-32 Nylon-Insert Thin Hex Locknut:59
- Insert:259: 45 Degree Gusset:2 ↔ Screw 8-32 x 0.375_:22
- Insert:260: 45 Degree Gusset:6 ↔ 8-32 Nylon-Insert Thin Hex Locknut:60
- Insert:263: Aluminum Angle 2x2x30:2 ↔ Aluminum C-Channel 1x2x1x12:4
- Insert:264: Aluminum Angle 2x2x30:2 ↔ Aluminum C-Channel 1x2x1x12:4
- Insert:265: Aluminum Angle 2x2x30:1 ↔ Aluminum C-Channel 1x2x1x12:4
- Insert:266: Aluminum Angle 2x2x30:1 ↔ Aluminum C-Channel 1x2x1x12:4
- Insert:267: Aluminum Angle 2x2x30:2 ↔ Aluminum C-Channel 1x2x1x12:5
- Insert:268: Aluminum Angle 2x2x30:2 ↔ Aluminum C-Channel 1x2x1x12:5
- Insert:269: Aluminum Angle 2x2x30:1 ↔ Aluminum C-Channel 1x2x1x12:5
- Insert:270: Aluminum Angle 2x2x30:1 ↔ Aluminum C-Channel 1x2x1x12:5
- Insert:271: Standoff 1.00_:5 ↔ Aluminum C-Channel 1x2x1x12:5
- Insert:272: Standoff 1.00_:6 ↔ Aluminum C-Channel 1x2x1x12:5
- Insert:273: Aluminum C-Channel 1x2x1x12:4 ↔ Standoff 1.00_:8
- Insert:274: Aluminum C-Channel 1x2x1x12:4 ↔ Standoff 1.00_:7
- Insert:279: Aluminum Angle 2x2x30:1 ↔ 45 Degree Gusset:9
- Insert:280: Aluminum Angle 2x2x30:1 ↔ 45 Degree Gusset:9
- Insert:281: Washer, Steel, 0.032_:9 ↔ 45 Degree Gusset:9
- Insert:282: Washer, Steel, 0.032_:9 ↔ Washer, Steel, 0.032_:10
- Insert:283: Aluminum Angle 2x2x30:2 ↔ 45 Degree Gusset:10
- Insert:284: Aluminum Angle 2x2x30:2 ↔ 45 Degree Gusset:10
- Insert:285: 45 Degree Gusset:3 ↔ Washer, Steel, 0.032_:10
- Insert:286: 45 Degree Gusset:10 ↔ Washer, Steel, 0.032_:11
- Insert:287: Washer, Steel, 0.032_:11 ↔ Washer, Steel, 0.032_:12
- Insert:288: 45 Degree Gusset:4 ↔ Washer, Steel, 0.032_:12
- Insert:289: 45 Degree Gusset:9 ↔ Screw 8-32 x 0.375_:23
- Insert:290: 45 Degree Gusset:9 ↔ Screw 8-32 x 0.375_:24
- Insert:291: 45 Degree Gusset:10 ↔ Screw 8-32 x 0.375_:25
- Insert:292: 45 Degree Gusset:10 ↔ Screw 8-32 x 0.375_:26
- Insert:293: 45 Degree Gusset:10 ↔ Screw 8-32 x 0.375_:27
- Insert:294: 45 Degree Gusset:9 ↔ Screw 8-32 x 0.375_:28
- Insert:295: 45 Degree Gusset:3 ↔ 8-32 Nylon-Insert Thin Hex Locknut:61
- Insert:296: Aluminum Angle 2x2x30:1 ↔ 8-32 Nylon-Insert Thin Hex Locknut:62
- Insert:297: Aluminum Angle 2x2x30:1 ↔ 8-32 Nylon-Insert Thin Hex Locknut:63
- Insert:298: 45 Degree Gusset:4 ↔ 8-32 Nylon-Insert Thin Hex Locknut:64
- Insert:299: Aluminum Angle 2x2x30:2 ↔ 8-32 Nylon-Insert Thin Hex Locknut:65
- Insert:300: Aluminum Angle 2x2x30:2 ↔ 8-32 Nylon-Insert Thin Hex Locknut:66
- Insert:301: Aluminum Angle 2x2x30:1 ↔ Screw 8-32 x 0.375_:29
- Insert:302: Aluminum Angle 2x2x30:1 ↔ Screw 8-32 x 0.375_:30
- Insert:303: Aluminum Angle 2x2x30:2 ↔ Screw 8-32 x 0.375_:31
- Insert:304: Aluminum Angle 2x2x30:2 ↔ Screw 8-32 x 0.375_:32
- Insert:305: Aluminum Angle 2x2x30:1 ↔ 8-32 Shoulder Screw:8
- Insert:306: Aluminum Angle 2x2x30:2 ↔ 8-32 Shoulder Screw:9
- Insert:307: Aluminum Angle 2x2x30:2 ↔ Screw 8-32 x 0.375_:33
- Insert:308: Aluminum Angle 2x2x30:1 ↔ Screw 8-32 x 0.375_:34
- Insert:309: Aluminum C-Channel 1x2x1x12:5 ↔ 8-32 Nylon-Insert Thin Hex Locknut:67
- Insert:310: Aluminum C-Channel 1x2x1x12:5 ↔ 8-32 Nylon-Insert Thin Hex Locknut:68
- Insert:311: Aluminum C-Channel 1x2x1x12:5 ↔ 8-32 Nylon-Insert Thin Hex Locknut:69
- Insert:312: Aluminum C-Channel 1x2x1x12:5 ↔ 8-32 Nylon-Insert Thin Hex Locknut:70
- Insert:313: Aluminum C-Channel 1x2x1x12:4 ↔ 8-32 Nylon-Insert Thin Hex Locknut:71
- Insert:314: Aluminum C-Channel 1x2x1x12:4 ↔ 8-32 Nylon-Insert Thin Hex Locknut:72
- Insert:315: Aluminum C-Channel 1x2x1x12:4 ↔ 8-32 Nylon-Insert Thin Hex Locknut:73
- Insert:316: Aluminum C-Channel 1x2x1x12:4 ↔ 8-32 Nylon-Insert Thin Hex Locknut:74
- Insert:317: Aluminum Angle 2x2x20:1 ↔ Aluminum C-Channel 1x2x1x12:6
- Insert:318: Aluminum Angle 2x2x20:1 ↔ Aluminum C-Channel 1x2x1x12:6
- Insert:319: Aluminum Angle 2x2x20:2 ↔ Aluminum C-Channel 1x2x1x12:6
- Insert:320: Aluminum Angle 2x2x20:2 ↔ Aluminum C-Channel 1x2x1x12:6
## Named parameters: d55_d51 = 0 mm, d56_d50 = 0 mm, d57_d48 = 0 mm, d58_d49 = 0 mm, d63_d41 = 0 mm, d64_d40 = 0 mm
